# Autodesk Inventor assembly: 090 ASY bottom
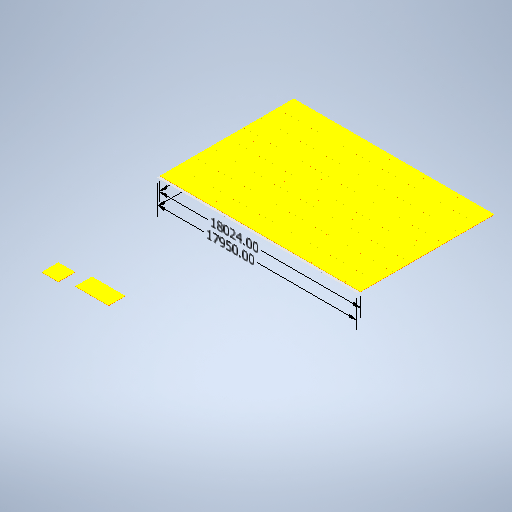
[picture p0: Inventor's stored thumbnail of the model, 512x512]
Saved by Autodesk Inventor 2026 (Build 300175000, 175)
## iProperties
Created: 2026-05-19
Part Number: 090 ASY bottom
Document SubType Name: Assembly
Designer: user
Author: user
## Documents named in this file (8)
- C:\Users\user\Documents\Inventor\GBK-Gubkinskiy\090 ASY bottom.iam
- C:\Users\user\Documents\Inventor\GBK-Gubkinskiy\0910.ipt
- C:\Users\user\Documents\Inventor\GBK-Gubkinskiy\092.iam
- C:\Users\user\Documents\Inventor\GBK-Gubkinskiy\093.iam
- C:\Users\user\Documents\Inventor\GBK-Gubkinskiy\092_CPY.iam
- C:\Users\user\Documents\Inventor\GBK-Gubkinskiy\093_CPY.iam
- C:\Users\user\Documents\Inventor\GBK-Gubkinskiy\092_CPY1.iam
- C:\Users\user\Documents\Inventor\GBK-Gubkinskiy\093_CPY1.iam
## Components (55 placed, 7 different names)
1. 0910:1 — Заподлицо:1, Заподлицо:2, Жесткий:1
2. 092:1 [sub-assembly] — Заподлицо:1
3. 093:1 [sub-assembly] — Заподлицо:2
4. 093_CPY:1 [sub-assembly] — Заподлицо:3, Заподлицо:4, Совмещение:1, Заподлицо:5, Заподлицо:6, Совмещение:2
5. 093_CPY1:1 [sub-assembly] — Заподлицо:7, Заподлицо:8, Совмещение:3
6. 093_CPY:2 [sub-assembly]
7. 093_CPY1:2 [sub-assembly]
8. 093_CPY:3 [sub-assembly]
9. 093_CPY1:3 [sub-assembly]
10. 093_CPY:4 [sub-assembly]
11. 093_CPY1:4 [sub-assembly]
12. 092_CPY:1 [sub-assembly] — Жесткий:1, Заподлицо:3, Заподлицо:4, Совмещение:1
13. 092_CPY:2 [sub-assembly]
14. 092_CPY:3 [sub-assembly]
15. 092_CPY:4 [sub-assembly]
16. 092_CPY:5 [sub-assembly]
17. 092_CPY:6 [sub-assembly]
18. 092_CPY:7 [sub-assembly]
19. 092_CPY:8 [sub-assembly]
20. 092_CPY:9 [sub-assembly]
21. 092_CPY:10 [sub-assembly]
22. 092_CPY:11 [sub-assembly]
23. 092_CPY:12 [sub-assembly]
24. 092_CPY:13 [sub-assembly]
25. 092_CPY:14 [sub-assembly]
26. 092_CPY:15 [sub-assembly]
27. 092_CPY:16 [sub-assembly]
28. 092_CPY:17 [sub-assembly]
29. 092_CPY:18 [sub-assembly]
30. 092_CPY:19 [sub-assembly]
31. 092_CPY:20 [sub-assembly]
32. 092_CPY:21 [sub-assembly]
33. 092_CPY:22 [sub-assembly]
34. 092_CPY:23 [sub-assembly]
35. 092_CPY:24 [sub-assembly]
36. 092_CPY1:1 [sub-assembly] — Заподлицо:5, Заподлицо:6, Совмещение:2
37. 092_CPY1:2 [sub-assembly]
38. 092_CPY1:3 [sub-assembly]
39. 092_CPY1:4 [sub-assembly]
40. 092_CPY1:5 [sub-assembly] — Заподлицо:7, Заподлицо:8, Совмещение:3
41. 092_CPY1:6 [sub-assembly]
42. 092_CPY1:7 [sub-assembly]
43. 092_CPY1:8 [sub-assembly]
44. 092_CPY1:9 [sub-assembly]
45. 092_CPY1:10 [sub-assembly]
46. 092_CPY1:11 [sub-assembly]
47. 092_CPY1:12 [sub-assembly]
48. 092_CPY1:13 [sub-assembly]
49. 092_CPY1:14 [sub-assembly]
50. 092_CPY1:15 [sub-assembly]
51. 092_CPY1:16 [sub-assembly]
52. 092_CPY1:17 [sub-assembly]
53. 092_CPY1:18 [sub-assembly]
54. 092_CPY1:19 [sub-assembly]
55. 092_CPY1:20 [sub-assembly]
## Component patterns: (4 elements), (4 elements, first: 093_CPY:1 + 093_CPY1:1), (6 elements, first: 092_CPY:1), МассивКомп 1:2 (6 elements), МассивКомп 1:3 (6 elements), МассивКомп 1:4 (6 elements), (5 elements, first: 092_CPY1:1), МассивКомп 2:2 (5 elements), МассивКомп 2:3 (5 elements), МассивКомп 2:4 (5 elements)
## Relationships (12: Flush 8, Mate 3, WeldJoint 1)
- Заподлицо:1 [Flush]: 0910:1 ↔ 092:1
- Заподлицо:2 [Flush]: 0910:1 ↔ 093:1
- Жесткий:1 [WeldJoint] (10 mm): 0910:1 ↔ 092_CPY:1
- Заподлицо:3 [Flush]: 093_CPY:1 ↔ 092_CPY:1
- Заподлицо:4 [Flush]: 093_CPY:1 ↔ 092_CPY:1
- Совмещение:1 [Mate] (4 mm): 093_CPY:1 ↔ 092_CPY:1
- Заподлицо:5 [Flush]: 093_CPY:1 ↔ 092_CPY1:1
- Заподлицо:6 [Flush]: 093_CPY:1 ↔ 092_CPY1:1
- Совмещение:2 [Mate] (4 mm): 093_CPY:1 ↔ 092_CPY1:1
- Заподлицо:7 [Flush]: 093_CPY1:1 ↔ 092_CPY1:5
- Заподлицо:8 [Flush]: 093_CPY1:1 ↔ 092_CPY1:5
- Совмещение:3 [Mate]: 093_CPY1:1 ↔ 092_CPY1:5
